# Autodesk Inventor assembly: Hex Interface Bearing
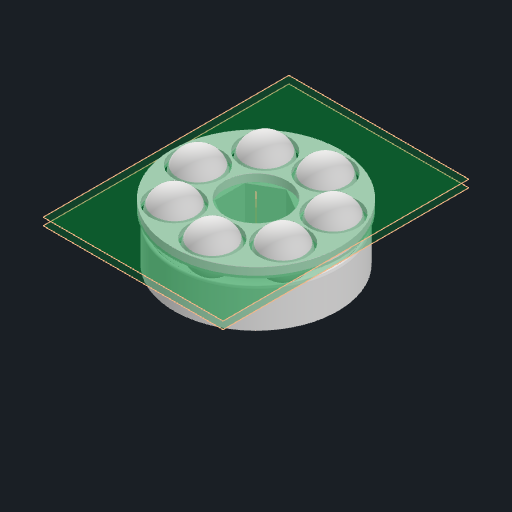
[picture p0: Inventor's stored thumbnail of the model, 512x512]
Saved by Autodesk Inventor 2023 (Build 270158000, 158)
## iProperties
Created: 2022-10-05
Part Number: Hex Interface Bearing
Document SubType Name: Assembly
Designer: izack
Author: izack
## Documents named in this file (4)
- E:\CAD Modeling\Private Robotics\Custom Tryhard Robot\Drivetrain\Swerve Module Parts\Hex Interface Bearing.iam
- E:\CAD Modeling\Private Robotics\Custom Tryhard Robot\Drivetrain\Swerve Module Parts\Hex Bearing Insert Parts\5mm Hex Bearing Interface.ipt
- E:\CAD Modeling\Private Robotics\Custom Tryhard Robot\Drivetrain\Swerve Module Parts\Hex Bearing Insert Parts\4.5mm Ball Bearings.ipt
- E:\CAD Modeling\Private Robotics\Custom Tryhard Robot\Drivetrain\Swerve Module Parts\Hex Bearing Insert Parts\Ball Bearing Spacer.ipt
## Components (9 placed, 3 different names)
1. 5mm Hex Bearing Interface:1 — Mate:1, Flush:1, Flush:2
2. Ball Bearing Spacer:1 — Flush:1, Flush:2
3. 4.5mm Ball Bearings:1 — Mate:1
4. 4.5mm Ball Bearings:2
5. 4.5mm Ball Bearings:3
6. 4.5mm Ball Bearings:4
7. 4.5mm Ball Bearings:5
8. 4.5mm Ball Bearings:6
9. 4.5mm Ball Bearings:7
## Component patterns: (7 elements, first: 4.5mm Ball Bearings:1)
## Relationships (3: Flush 2, Mate 1)
- Mate:1 (5.85 mm): 5mm Hex Bearing Interface:1 ↔ 4.5mm Ball Bearings:1
- Flush:1 (-5.75 mm): 5mm Hex Bearing Interface:1 ↔ Ball Bearing Spacer:1
- Flush:2 (-5 mm): 5mm Hex Bearing Interface:1 ↔ Ball Bearing Spacer:1
